# Autodesk Inventor assembly: testasm1
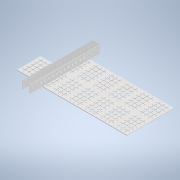
[picture p0: Inventor's stored thumbnail of the model, 180x180]
Saved by Autodesk Inventor 2020.1 (Build 241239000, 239)
## iProperties
Created: 2019-12-07
Part Number: testasm1
Document SubType Name: Assembly
Designer: tbloo
Author: tbloo
## Documents named in this file (3)
- B:\Documents\GitHub\AO_Robotics\CAD\Projects\Timothy Bloot\Tango\testasm1.iam
- B:\Documents\GitHub\AO_Robotics\CAD\Projects\Timothy Bloot\Tango\spacerplate.ipt
- B:\Documents\GitHub\AO_Robotics\CAD\Parts Kits\FTC Tetrix KOP Organized (7-24-19)\Frame Hardware\Tetrix_39068.ipt
## Components (14 placed, 2 different names)
1. spacerplate:1 — Mate:11, Flush:21, Flush:22
2. spacerplate:2
3. spacerplate:3
4. spacerplate:4
5. spacerplate:5
6. spacerplate:6
7. spacerplate:7
8. spacerplate:8
9. spacerplate:9 — Mate:11, Flush:21, Flush:22
10. spacerplate:10
11. spacerplate:11
12. spacerplate:12
13. spacerplate:13
14. Tetrix_39068:1
## Relationships (33: Flush 22, Mate 11)
- [Flush]: spacerplate:1 ↔ spacerplate:2
- [Flush]: spacerplate:1 ↔ spacerplate:2
- [Mate]: spacerplate:1 ↔ spacerplate:2
- [Flush]: spacerplate:2 ↔ spacerplate:3
- [Flush]: spacerplate:2 ↔ spacerplate:3
- [Mate]: spacerplate:2 ↔ spacerplate:3
- [Flush]: spacerplate:4 ↔ spacerplate:5
- [Flush]: spacerplate:4 ↔ spacerplate:5
- [Mate]: spacerplate:4 ↔ spacerplate:5
- [Flush]: spacerplate:5 ↔ spacerplate:6
- [Flush]: spacerplate:5 ↔ spacerplate:6
- [Mate]: spacerplate:5 ↔ spacerplate:6
- [Mate]: spacerplate:2 ↔ spacerplate:6
- [Flush]: spacerplate:1 ↔ spacerplate:6
- [Flush]: spacerplate:3 ↔ spacerplate:6
- [Flush]: spacerplate:7 ↔ spacerplate:8
- [Flush]: spacerplate:7 ↔ spacerplate:8
- [Mate]: spacerplate:7 ↔ spacerplate:8
- [Flush]: spacerplate:8 ↔ spacerplate:9
- [Flush]: spacerplate:8 ↔ spacerplate:9
- [Mate]: spacerplate:8 ↔ spacerplate:9
- [Flush]: spacerplate:10 ↔ spacerplate:11
- [Flush]: spacerplate:10 ↔ spacerplate:11
- [Mate]: spacerplate:10 ↔ spacerplate:11
- [Flush]: spacerplate:11 ↔ spacerplate:12
- [Flush]: spacerplate:11 ↔ spacerplate:12
- [Mate]: spacerplate:11 ↔ spacerplate:12
- [Mate]: spacerplate:8 ↔ spacerplate:12
- [Flush]: spacerplate:7 ↔ spacerplate:12
- [Flush]: spacerplate:9 ↔ spacerplate:12
- Mate:11: spacerplate:1 ↔ spacerplate:9
- Flush:21: spacerplate:1 ↔ spacerplate:9
- Flush:22: spacerplate:1 ↔ spacerplate:9
## Named parameters: d204_d197 = 0 mm, d205_d198 = 0 mm, d206_d199 = 0 mm, d207_d200 = 0 mm, d208_d201 = 0 mm, d209_d202 = 0 mm, d15_d210 = 0 mm, d16_d211 = 0 mm, d17_d212 = 0 mm, d18_d197 = 0 mm, d19_d198 = 0 mm, d20_d199 = 0 mm, d21_d200 = 0 mm, d22_d201 = 0 mm, d23_d202 = 0 mm, d24_d204_d197 = 0 mm, d25_d205_d198 = 0 mm, d26_d206_d199 = 0 mm, d27_d207_d200 = 0 mm, d28_d208_d201 = 0 mm, d29_d209_d202 = 0 mm
